# Autodesk Inventor assembly: ASY PNS-Filter column D1200
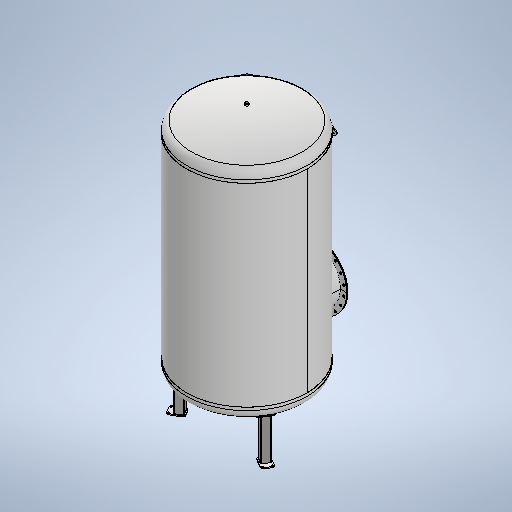
[picture p0: Inventor's stored thumbnail of the model, 512x512]
Saved by Autodesk Inventor 2025 (Build 290162010, 162A)
## iProperties
Created: 2025-02-13
Part Number: ASY PNS-Filter column D1200
Document SubType Name: Assembly
Designer: pokla
Author: pokla
Revision Number: 3
## Documents named in this file (15)
- C:\Users\admin\YandexDisk-badmisterfox\home pc\Inventor\PNS-Panaevsk\D1000\ASY PNS-Filter column D1200.iam
- C:\Users\admin\YandexDisk-badmisterfox\home pc\Inventor\PNS-Panaevsk\Filter D1200\PNS-721 charging hatch D1200.ipt
- C:\Users\admin\YandexDisk-badmisterfox\home pc\Inventor\PNS-Panaevsk\Filter D1200\PNS-712 accses hatch flangeipt.ipt
- C:\Users\admin\YandexDisk-badmisterfox\home pc\Inventor\PNS-Panaevsk\Filter D1200\000 DIM PNS-Filter column D1200.ipt
- C:\Users\admin\YandexDisk-badmisterfox\home pc\Inventor\PNS-Panaevsk\Filter D1200\PNS-711 accses hatch tube.ipt
- C:\Users\admin\YandexDisk-badmisterfox\home pc\Inventor\PNS-Panaevsk\Filter D1200\PNS-701 main tube D1200.ipt
- C:\Users\admin\YandexDisk-badmisterfox\home pc\Inventor\PNS-Panaevsk\Filter D1200\PNS- 752 tube.ipt
- C:\Users\admin\YandexDisk-badmisterfox\home pc\Inventor\PNS-Panaevsk\Filter D1200\PNV - 704 dished head D1200.ipt
- C:\Users\admin\YandexDisk-badmisterfox\home pc\Inventor\PNS-Panaevsk\D1000\Fitting G1.ipt
- C:\Users\admin\YandexDisk-badmisterfox\home pc\Inventor\PNS-Panaevsk\Filter D1200\PNS- 723 charging half tube.ipt
- C:\Users\admin\YandexDisk-badmisterfox\home pc\Inventor\PNS-Panaevsk\CC\en-US\DIN 2576 PN 10(2)\DIN 2576 Slip-On Flange for Welding Series 1 (ISO) - PN 10 500 x 508.ipt
- C:\Users\admin\YandexDisk-badmisterfox\home pc\Inventor\PNS-Panaevsk\Filter D1200\ASY PNS780-Filter legs D1200.iam
- C:\Users\admin\YandexDisk-badmisterfox\home pc\Inventor\PNS-Panaevsk\CC\en-US\DIN 2576 PN 10(2)\DIN 2576 Slip-On Flange for Welding Series 1 (ISO) - PN 10 80 x 88.9.ipt
- C:\Users\admin\YandexDisk-badmisterfox\home pc\Inventor\PNS-Panaevsk\Filter D1200\PNS-733 charging flange round.ipt
- C:\Users\admin\YandexDisk-badmisterfox\home pc\Inventor\PNS-Panaevsk\Filter D1200\sprinkler dummy.ipt
## Components (61 placed, 14 different names)
1. 000 DIM PNS-Filter column D1200.ipt:1
2. PNS-721 charging hatch D1200.ipt:1 — Rigid:29
3. PNS-712 accses hatch flangeipt.ipt:1 — Rigid:24, Rigid:25, Rigid:27, Rigid:28
4. PNS-711 accses hatch tube.ipt:1 — Rigid:10, Rigid:27
5. PNS-701 main tube D1200.ipt:1 — Rigid:10, Rigid:13, Rigid:14, Mate:1, Mate:2, Rigid:31, Rigid:33, Rigid:34
6. PNS- 752 tube.ipt:1 — Rotational:2, Rigid:33
7. PNS-712 accses hatch flangeipt.ipt:2 — Rigid:24, Rigid:26
8. PNS- 752 tube.ipt:2 — Rotational:1, Rigid:34
9. PNV - 704 dished head D1200.ipt:1 — Rigid:13, Rigid:16
10. PNV - 704 dished head D1200.ipt:2 — Rigid:14, Rigid:15, Mate:3
11. Fitting G1.ipt:1 — Rigid:15
12. Fitting G1.ipt:2 — Rigid:16
13. PNS- 723 charging half tube.ipt:2 — Rigid:31, Rigid:32
14. DIN 2576 Slip-On Flange for Welding Series 1 (ISO) - PN 10 500 x 508.ipt:1 — Rigid:28
15. PNS-712 accses hatch flangeipt.ipt:3 — Rigid:25, Rigid:29
16. PNS-712 accses hatch flangeipt.ipt:4 — Rigid:26
17. Assembly2.iam:1 [sub-assembly] — Flush:1, Flush:2, Flush:3
18. DIN 2576 Slip-On Flange for Welding Series 1 (ISO) - PN 10 80 x 88.9.ipt:1 — Rotational:2
19. DIN 2576 Slip-On Flange for Welding Series 1 (ISO) - PN 10 80 x 88.9.ipt:2 — Rotational:1
20. PNS-733 charging flange round:1 — Rigid:32
21. sprinkler dummy:1
22. sprinkler dummy:2
23. sprinkler dummy:3
24. sprinkler dummy:4
25. sprinkler dummy:5
26. sprinkler dummy:6
27. sprinkler dummy:7
28. sprinkler dummy:8
29. sprinkler dummy:9
30. sprinkler dummy:10
31. sprinkler dummy:11
32. sprinkler dummy:12
33. sprinkler dummy:13
34. sprinkler dummy:14
35. sprinkler dummy:15
36. sprinkler dummy:16
37. sprinkler dummy:17
38. sprinkler dummy:18
39. sprinkler dummy:19
40. sprinkler dummy:20
41. sprinkler dummy:21
42. sprinkler dummy:22
43. sprinkler dummy:23
44. sprinkler dummy:24
45. sprinkler dummy:25
46. sprinkler dummy:26
47. sprinkler dummy:27
48. sprinkler dummy:28
49. sprinkler dummy:29
50. sprinkler dummy:30
51. sprinkler dummy:31
52. sprinkler dummy:32
53. sprinkler dummy:33
54. sprinkler dummy:34
55. sprinkler dummy:35
56. sprinkler dummy:36
57. sprinkler dummy:37
58. sprinkler dummy:38
59. sprinkler dummy:39
60. sprinkler dummy:40
61. sprinkler dummy:41
## Relationships (23: WeldJoint 15, Mate 3, Flush 3, RevoluteJoint 2)
- Rigid:10 [WeldJoint] (66 mm): PNS-711 accses hatch tube.ipt:1 ↔ PNS-701 main tube D1200.ipt:1
- Rigid:13 [WeldJoint]: PNS-701 main tube D1200.ipt:1 ↔ PNV - 704 dished head D1200.ipt:1
- Rigid:14 [WeldJoint]: PNS-701 main tube D1200.ipt:1 ↔ PNV - 704 dished head D1200.ipt:2
- Rigid:15 [WeldJoint]: PNV - 704 dished head D1200.ipt:2 ↔ Fitting G1.ipt:1
- Rigid:16 [WeldJoint]: PNV - 704 dished head D1200.ipt:1 ↔ Fitting G1.ipt:2
- Rigid:24 [WeldJoint]: PNS-712 accses hatch flangeipt.ipt:1 ↔ PNS-712 accses hatch flangeipt.ipt:2
- Rigid:25 [WeldJoint]: PNS-712 accses hatch flangeipt.ipt:1 ↔ PNS-712 accses hatch flangeipt.ipt:3
- Rigid:26 [WeldJoint]: PNS-712 accses hatch flangeipt.ipt:2 ↔ PNS-712 accses hatch flangeipt.ipt:4
- Rigid:27 [WeldJoint]: PNS-712 accses hatch flangeipt.ipt:1 ↔ PNS-711 accses hatch tube.ipt:1
- Rigid:28 [WeldJoint]: PNS-712 accses hatch flangeipt.ipt:1 ↔ DIN 2576 Slip-On Flange for Welding Series 1 (ISO) - PN 10 500 x 508.ipt:1
- Mate:1: PNS-701 main tube D1200.ipt:1
- Mate:2: PNS-701 main tube D1200.ipt:1
- Mate:3 (2750 mm): PNV - 704 dished head D1200.ipt:2
- Flush:1: Assembly2.iam:1
- Flush:2: Assembly2.iam:1
- Flush:3: Assembly2.iam:1
- Rigid:29 [WeldJoint]: PNS-721 charging hatch D1200.ipt:1 ↔ PNS-712 accses hatch flangeipt.ipt:3
- Rotational:1 [RevoluteJoint]: PNS- 752 tube.ipt:2 ↔ DIN 2576 Slip-On Flange for Welding Series 1 (ISO) - PN 10 80 x 88.9.ipt:2
- Rotational:2 [RevoluteJoint]: PNS- 752 tube.ipt:1 ↔ DIN 2576 Slip-On Flange for Welding Series 1 (ISO) - PN 10 80 x 88.9.ipt:1
- Rigid:31 [WeldJoint]: PNS-701 main tube D1200.ipt:1 ↔ PNS- 723 charging half tube.ipt:2
- Rigid:32 [WeldJoint]: PNS- 723 charging half tube.ipt:2 ↔ PNS-733 charging flange round:1
- Rigid:33 [WeldJoint]: PNS-701 main tube D1200.ipt:1 ↔ PNS- 752 tube.ipt:1
- Rigid:34 [WeldJoint]: PNS-701 main tube D1200.ipt:1 ↔ PNS- 752 tube.ipt:2
